# Autodesk Inventor assembly: GA_Assembly
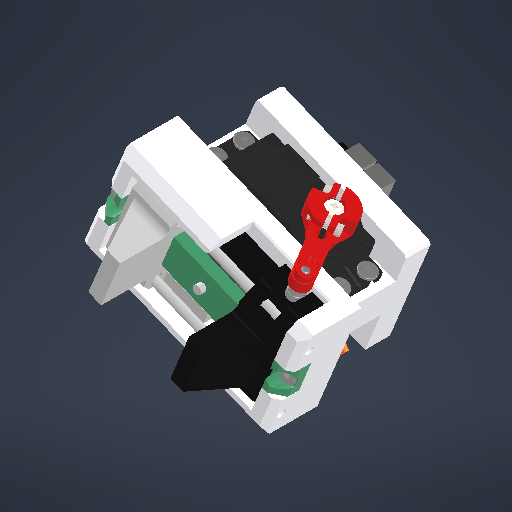
[picture p0: Inventor's stored thumbnail of the model, 512x512]
Saved by Autodesk Inventor 2025.2 (Build 292293000, 293)
## iProperties
Created: 2025-07-02
Part Number: GA_Assembly
Document SubType Name: Assembly
Designer: Tiago
Author: Tiago
## Documents named in this file (16)
- C:\Users\Tiago\Documents\Inventor\Exp. Braço v1\GA_Assembly.iam
- C:\Users\Tiago\Documents\Inventor\Exp. Braço v1\GA_Base.ipt
- C:\Users\Tiago\Documents\Inventor\Exp. Braço v1\GA_Engrenagem.ipt
- C:\Users\Tiago\Documents\Inventor\Exp. Braço v1\GA_FixaBase.ipt
- C:\Users\Tiago\Documents\Inventor\Exp. Braço v1\GA_veioD3_L17.ipt
- C:\Users\Tiago\Documents\Inventor\Exp. Braço v1\GA_2.ipt
- C:\Users\Tiago\Documents\Inventor\Exp. Braço v1\GA_1.ipt
- C:\Users\Tiago\Documents\Inventor\Exp. Braço v1\GA_veioD3_L70.ipt
- C:\Users\Tiago\Documents\Inventor\Exp. Braço v1\Linear_Shaft_Support_SHF8.ipt
- C:\Users\Tiago\Documents\Inventor\Exp. Braço v1\M5x16L_Hex.ipt
- C:\Users\Tiago\Documents\Inventor\Exp. Braço v1\M5_nylonLock_Nut.ipt
- C:\Users\Tiago\Documents\Inventor\Exp. Braço v1\M3 x0.5 ALT (...).ipt
- C:\Users\Tiago\Documents\Inventor\Exp. Braço v1\MG996R_Servo_Motor_WithHorn.iam
- C:\Users\Tiago\Documents\Inventor\Exp. Braço v1\M3 x8L_hexagonal_BigHEAD.ipt
- C:\Users\Tiago\Documents\Inventor\Exp. Braço v1\M5 x12L_Hex_C.ipt
- M5 x12L_Hex_C.ipt
## Components (22 placed, 14 different names)
1. GA_Base:1 — Mate:1, Mate:2, Mate:3, Mate:4, Mate:6, Mate:7, Mate:8, Mate:9, Mate:10, Mate:11, Flush:1, Mate:12, Mate:13, Mate:14, Mate:15, Flush:2, Mate:16, Mate:17, Mate:18, Insert:3, Insert:4, Mate:19, Mate:20, Mate:21
2. GA_Engrenagem:1 — Mate:5, Mate:6
3. GA_FixaBase:1 — Mate:11, Flush:1, Mate:12, Insert:5, Insert:6
4. GA_veioD3_L17:1 — Mate:3, Mate:4, Mate:5
5. GA_2:1 — Mate:9, Mate:10
6. GA_1:1 — Mate:7, Mate:8
7. GA_veioD3_L70:1 — Mate:13, Mate:15
8. GA_veioD3_L70:2 — Mate:14, Flush:2
9. Linear_Shaft_Support_SHF8:1 — Mate:16, Mate:17, Mate:18, Insert:1, Insert:2, Insert:11
10. M5x16L_Hex:1 — Insert:2
11. M5x16L_Hex:2 — Insert:1
12. M5_nylonLock_Nut:1 — Insert:4
13. M5_nylonLock_Nut:2 — Insert:3
14. M3 x0.5 ALT (...):1 — Insert:5
15. M3 x0.5 ALT (...):2 — Insert:6
16. MG996R_Servo_Motor_WithHorn:1 [sub-assembly] — Mate:19, Mate:20, Mate:21, Insert:7, Insert:8, Insert:9, Insert:10, Mate:22, Mate:23
17. M3 x8L_hexagonal_BigHEAD:1 — Mate:22, Mate:23
18. M3 x0.5 ALT (...):3 — Insert:8
19. M3 x0.5 ALT (...):4 — Insert:7
20. M3 x0.5 ALT (...):5 — Insert:9
21. M3 x0.5 ALT (...):6 — Insert:10
22. M5 x12L_Hex_C:1 — Insert:11
## Relationships (36: Mate 23, Insert 11, Flush 2)
- Mate:1: GA_Base:1
- Mate:2: GA_Base:1
- Mate:3: GA_Base:1 ↔ GA_veioD3_L17:1
- Mate:4: GA_Base:1 ↔ GA_veioD3_L17:1
- Mate:5: GA_Engrenagem:1 ↔ GA_veioD3_L17:1
- Mate:6 (0.5 mm): GA_Base:1 ↔ GA_Engrenagem:1
- Mate:7: GA_Base:1 ↔ GA_1:1
- Mate:8: GA_Base:1 ↔ GA_1:1
- Mate:9: GA_Base:1 ↔ GA_2:1
- Mate:10: GA_Base:1 ↔ GA_2:1
- Mate:11: GA_Base:1 ↔ GA_FixaBase:1
- Flush:1: GA_Base:1 ↔ GA_FixaBase:1
- Mate:12: GA_Base:1 ↔ GA_FixaBase:1
- Mate:13: GA_Base:1 ↔ GA_veioD3_L70:1
- Mate:14: GA_Base:1 ↔ GA_veioD3_L70:2
- Mate:15 (-1 mm): GA_Base:1 ↔ GA_veioD3_L70:1
- Flush:2 (1 mm): GA_Base:1 ↔ GA_veioD3_L70:2
- Mate:16: GA_Base:1 ↔ Linear_Shaft_Support_SHF8:1
- Mate:17: GA_Base:1 ↔ Linear_Shaft_Support_SHF8:1
- Mate:18: GA_Base:1 ↔ Linear_Shaft_Support_SHF8:1
- Insert:1: Linear_Shaft_Support_SHF8:1 ↔ M5x16L_Hex:2
- Insert:2: Linear_Shaft_Support_SHF8:1 ↔ M5x16L_Hex:1
- Insert:3: GA_Base:1 ↔ M5_nylonLock_Nut:2
- Insert:4: GA_Base:1 ↔ M5_nylonLock_Nut:1
- Insert:5: GA_FixaBase:1 ↔ M3 x0.5 ALT (...):1
- Insert:6: GA_FixaBase:1 ↔ M3 x0.5 ALT (...):2
- Mate:19: GA_Base:1 ↔ MG996R_Servo_Motor_WithHorn:1
- Mate:20: GA_Base:1 ↔ MG996R_Servo_Motor_WithHorn:1
- Mate:21: GA_Base:1 ↔ MG996R_Servo_Motor_WithHorn:1
- Insert:7: MG996R_Servo_Motor_WithHorn:1 ↔ M3 x0.5 ALT (...):4
- Insert:8: MG996R_Servo_Motor_WithHorn:1 ↔ M3 x0.5 ALT (...):3
- Insert:9: MG996R_Servo_Motor_WithHorn:1 ↔ M3 x0.5 ALT (...):5
- Insert:10: MG996R_Servo_Motor_WithHorn:1 ↔ M3 x0.5 ALT (...):6
- Mate:22 (2 mm): MG996R_Servo_Motor_WithHorn:1 ↔ M3 x8L_hexagonal_BigHEAD:1
- Mate:23: MG996R_Servo_Motor_WithHorn:1 ↔ M3 x8L_hexagonal_BigHEAD:1
- Insert:11: Linear_Shaft_Support_SHF8:1 ↔ M5 x12L_Hex_C:1
